# Autodesk Inventor assembly: Induction Motor
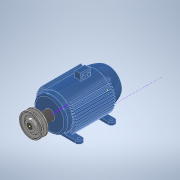
[picture p0: Inventor's stored thumbnail of the model, 180x180]
Saved by Autodesk Inventor 2021 (Build 250183000, 183)
## iProperties
Created: 2021-07-30
Part Number: Induction Motor
Document SubType Name: Assembly
Designer: MOGIRE
Author: MOGIRE
## Documents named in this file (5)
- C:\Users\MOGIRE\Documents\Manufacturing Technology 4.1\Induction Motor.iam
- C:\Users\MOGIRE\Documents\Manufacturing Technology 4.1\Motor_Frame_.ipt
- C:\Users\MOGIRE\Documents\Manufacturing Technology 4.1\Fan_cover_1.ipt
- C:\Users\MOGIRE\Documents\Manufacturing Technology 4.1\Squirrel cage.ipt
- C:\Users\MOGIRE\Documents\Manufacturing Technology 4.1\Pulley.ipt
## Components (4 placed, 4 different names)
1. Motor_Frame_:1 — Mate:1, Mate:2, Mate:3, Flush:1, Mate:4
2. Fan_cover_1:1 — Mate:2, Mate:3
3. Squirrel cage:1 — Flush:1, Mate:4, Mate:5, Mate:6
4. Pulley:1 — Mate:5, Mate:6
## Relationships (7: Mate 6, Flush 1)
- Mate:1: Motor_Frame_:1
- Mate:2: Motor_Frame_:1 ↔ Fan_cover_1:1
- Mate:3: Motor_Frame_:1 ↔ Fan_cover_1:1
- Flush:1 (50 mm): Motor_Frame_:1 ↔ Squirrel cage:1
- Mate:4: Motor_Frame_:1 ↔ Squirrel cage:1
- Mate:5 (20 mm): Squirrel cage:1 ↔ Pulley:1
- Mate:6: Squirrel cage:1 ↔ Pulley:1
